# Autodesk Inventor assembly: tailpipe assembly
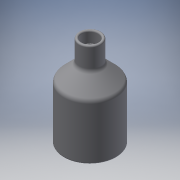
[picture p0: Inventor's stored thumbnail of the model, 180x180]
Saved by Autodesk Inventor 2016 (Build 200138000, 138)
## iProperties
Created: 2015-08-17
Part Number: tailpipe assembly
Document SubType Name: Assembly
## Documents named in this file (3)
- C:\Users\charlie\Documents\Inventor\Car Parts\Tailpipe\tailpipe assembly.iam
- C:\Users\charlie\Documents\Inventor\Car Parts\Tailpipe\tailpipe.ipt
- C:\Users\charlie\Documents\Inventor\Car Parts\Tailpipe\insert.ipt
## Components (2 placed, 2 different names)
1. tailpipe:1 — Insert:1
2. insert:1 — Insert:1
## Relationships (1: Insert 1)
- Insert:1 (9 mm): tailpipe:1 ↔ insert:1
